# Autodesk Inventor assembly: ridgidity analysis2
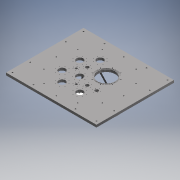
[picture p0: Inventor's stored thumbnail of the model, 180x180]
Saved by Autodesk Inventor 2018 (Build 220112000, 112)
## iProperties
Created: 2019-01-14
Part Number: ridgidity analysis2
Document SubType Name: Assembly
Designer: Admin
Author: Admin
## Documents named in this file (4)
- C:\Users\Admin\Documents\Cryostat\CAD\ridgidity analysis2.iam
- C:\Users\Admin\Documents\Cryostat\CAD\Top Plate V2.2.ipt
- C:\Users\Admin\Documents\Cryostat\CAD\foot type 3.iam
- C:\Users\Admin\Documents\Cryostat\CAD\mini 55K stage.ipt
## Components (10 placed, 3 different names)
1. Top Plate V2.2:1 — Mate:3, Mate:4, Mate:5, Mate:6, Mate:7, Mate:8, Mate:9, Mate:10, Mate:11, Mate:12, Mate:13, Mate:14, Mate:15, Mate:16, Mate:26, Mate:27
2. foot type 3:1 [sub-assembly] — Mate:12, Mate:25, Mate:26
3. foot type 3:2 [sub-assembly] — Mate:11, Mate:24, Mate:27
4. foot type 3:3 [sub-assembly] — Mate:3, Mate:15, Mate:23
5. foot type 3:4 [sub-assembly] — Mate:4, Mate:16, Mate:22
6. foot type 3:5 [sub-assembly] — Mate:5, Mate:13, Mate:20
7. foot type 3:6 [sub-assembly] — Mate:6, Mate:14, Mate:19, Mate:21
8. foot type 3:7 [sub-assembly] — Mate:7, Mate:10, Mate:18
9. foot type 3:8 [sub-assembly] — Mate:8, Mate:9, Mate:17
10. mini 55K stage:1 — Mate:17, Mate:18, Mate:19, Mate:20, Mate:21, Mate:22, Mate:23, Mate:24, Mate:25
## Relationships (25: Mate 25)
- Mate:3: Top Plate V2.2:1 ↔ foot type 3:3
- Mate:4: Top Plate V2.2:1 ↔ foot type 3:4
- Mate:5: Top Plate V2.2:1 ↔ foot type 3:5
- Mate:6: Top Plate V2.2:1 ↔ foot type 3:6
- Mate:7: Top Plate V2.2:1 ↔ foot type 3:7
- Mate:8: Top Plate V2.2:1 ↔ foot type 3:8
- Mate:9: Top Plate V2.2:1 ↔ foot type 3:8
- Mate:10: Top Plate V2.2:1 ↔ foot type 3:7
- Mate:11: Top Plate V2.2:1 ↔ foot type 3:2
- Mate:12: Top Plate V2.2:1 ↔ foot type 3:1
- Mate:13: Top Plate V2.2:1 ↔ foot type 3:5
- Mate:14: Top Plate V2.2:1 ↔ foot type 3:6
- Mate:15: Top Plate V2.2:1 ↔ foot type 3:3
- Mate:16: Top Plate V2.2:1 ↔ foot type 3:4
- Mate:17: foot type 3:8 ↔ mini 55K stage:1
- Mate:18: foot type 3:7 ↔ mini 55K stage:1
- Mate:19: foot type 3:6 ↔ mini 55K stage:1
- Mate:20: foot type 3:5 ↔ mini 55K stage:1
- Mate:21: foot type 3:6 ↔ mini 55K stage:1
- Mate:22: foot type 3:4 ↔ mini 55K stage:1
- Mate:23: foot type 3:3 ↔ mini 55K stage:1
- Mate:24: foot type 3:2 ↔ mini 55K stage:1
- Mate:25: foot type 3:1 ↔ mini 55K stage:1
- Mate:26: Top Plate V2.2:1 ↔ foot type 3:1
- Mate:27: Top Plate V2.2:1 ↔ foot type 3:2
